# Autodesk Inventor assembly: Drivebase AM14U4 Square 28inx28in v411
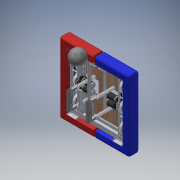
[picture p0: Inventor's stored thumbnail of the model, 180x180]
Saved by Autodesk Inventor 2018 (Build 220112000, 112)
## iProperties
Created: 2020-01-28
Part Number: Drivebase AM14U4 Square 28inx28in v411
Document SubType Name: Assembly
Designer: Weeb No1
Sending System: Autodesk Translation Framework v8.12.0.6
Preprocessor: ST-DEVELOPER v18
Title: /Users/GabG/Documents/GitHub/2020CAD/New Gabriel Shooter/Drivebase AM14U4 Square 28inx28in v41.step
## Documents named in this file (17)
- C:\Users\Weeb No1\Documents\GitHub\2020CAD\Gabriel Fixed Inventor Versions\Drivebase\Main Assembly\Drivebase AM14U4 Square 28inx28in v411.iam
- C:\Users\Weeb No1\Documents\GitHub\2020CAD\Gabriel Fixed Inventor Versions\Drivebase\Part Files\AM14U4 Square Half.iam
- C:\Users\Weeb No1\Documents\GitHub\2020CAD\Gabriel Fixed Inventor Versions\Drivebase\Part Files\AM14U4 Square Half_1.iam
- C:\Users\Weeb No1\Documents\GitHub\2020CAD\Gabriel Fixed Inventor Versions\Drivebase\Part Files\Placeholder Belly Pan.ipt
- C:\Users\Weeb No1\Documents\GitHub\2020CAD\Gabriel Fixed Inventor Versions\Drivebase\Part Files\10-24 Washer.ipt
- C:\Users\Weeb No1\Documents\GitHub\2020CAD\Gabriel Fixed Inventor Versions\Drivebase\Part Files\Bumper Assembly.iam
- C:\Users\Weeb No1\Documents\GitHub\2020CAD\Gabriel Fixed Inventor Versions\Drivebase\Part Files\Bumper Assembly_1.iam
- C:\Users\Weeb No1\Documents\GitHub\2020CAD\Gabriel Fixed Inventor Versions\Drivebase\Part Files\95335A503_METRIC QUICK-RELEASE PIN.ipt
- C:\Users\Weeb No1\Documents\GitHub\2020CAD\Gabriel Fixed Inventor Versions\Drivebase\Part Files\8020 1010 x 19 v2.ipt
- C:\Users\Weeb No1\Documents\GitHub\2020CAD\Gabriel Fixed Inventor Versions\Drivebase\Part Files\8020 1010 x 11 5 v2.ipt
- C:\Users\Weeb No1\Documents\GitHub\2020CAD\Gabriel Fixed Inventor Versions\Drivebase\Part Files\1x2 9in 1_16_ Beam v7.ipt
- C:\Users\Weeb No1\Documents\GitHub\2020CAD\Gabriel Fixed Inventor Versions\Drivebase\Part Files\L-Guesset v1.ipt
- C:\Users\Weeb No1\Documents\GitHub\2020CAD\Gabriel Fixed Inventor Versions\Drivebase\Part Files\L-Bracket v1.ipt
- C:\Users\Weeb No1\Documents\GitHub\2020CAD\Gabriel Fixed Inventor Versions\Drivebase\Part Files\Component52.ipt
- C:\Users\Weeb No1\Documents\GitHub\2020CAD\Gabriel Fixed Inventor Versions\Drivebase\Part Files\8020 1010 x 8 7_8 v6.ipt
- C:\Users\Weeb No1\Documents\GitHub\2020CAD\Gabriel Fixed Inventor Versions\Drivebase\Part Files\am-2986 FR8ZZ Hex Bearing v1.ipt
- C:\Users\Weeb No1\Documents\GitHub\2020CAD\Gabriel Fixed Inventor Versions\Drivebase\Part Files\Clamping_Shaft_Collar_-_1_2_Hex_ID_217-2737 v1.ipt
## Components (59 placed, 16 different names)
1. AM14U4 Square Half:1 [sub-assembly] — Mate:1, Flush:2, Flush:1, Mate:2, Flush:4, Flush:3
2. AM14U4 Square Half_1:1 [sub-assembly]
3. Placeholder Belly Pan:1 — Mate:21, Mate:59, Mate:22, Mate:58
4. 10-24 Washer:1
5. 10-24 Washer:2
6. 10-24 Washer:3
7. 10-24 Washer:4
8. 10-24 Washer:5
9. 10-24 Washer:6
10. 10-24 Washer:7
11. 10-24 Washer:8
12. Bumper Assembly:1 [sub-assembly]
13. Bumper Assembly_1:1 [sub-assembly]
14. 95335A503_METRIC QUICK-RELEASE PIN:1
15. 95335A503_METRIC QUICK-RELEASE PIN:2
16. 95335A503_METRIC QUICK-RELEASE PIN:3
17. 95335A503_METRIC QUICK-RELEASE PIN:4
18. 95335A503_METRIC QUICK-RELEASE PIN:5
19. 95335A503_METRIC QUICK-RELEASE PIN:6
20. 95335A503_METRIC QUICK-RELEASE PIN:7
21. 95335A503_METRIC QUICK-RELEASE PIN:8
22. 95335A503_METRIC QUICK-RELEASE PIN:9
23. 95335A503_METRIC QUICK-RELEASE PIN:10
24. 95335A503_METRIC QUICK-RELEASE PIN:11
25. 95335A503_METRIC QUICK-RELEASE PIN:12
26. 8020 1010 x 19 v2:1 — Mate:1, Flush:2, Flush:1, Flush:17, Mate:20, Mate:19
27. 8020 1010 x 19 v2:2 — Mate:2, Flush:4, Flush:3, Mate:60, Flush:41, Mate:61
28. 8020 1010 x 11 5 v2:1 — Mate:21, Flush:17, Mate:20, Mate:18, Flush:16, Flush:15, Flush:18, Mate:25
29. 8020 1010 x 11 5 v2:2 — Mate:60, Flush:41, Mate:59, Flush:39, Flush:38, Mate:56, Mate:55, Flush:23, Mate:32
30. 8020 1010 x 11 5 v2:3 — Mate:22, Mate:19, Flush:14, Flush:13, Mate:17, Flush:21, Mate:29
31. 1x2 9in 1_16_ Beam v7:1 — Mate:18, Flush:16, Flush:15, Flush:14, Flush:13, Mate:17, Mate:8, Mate:7, Mate:6, Flush:8, Flush:7, Mate:14, Mate:13, Mate:12, Flush:12, Flush:11, Flush:32, Flush:31, Mate:5, Mate:4, Mate:3, Flush:6, Flush:5, Mate:11, Mate:10, Mate:9, Flush:10, Flush:9, Mate:16, Mate:15
32. 8020 1010 x 11 5 v2:4 — Mate:61, Mate:58, Flush:40, Flush:37, Mate:57, Flush:28, Mate:37
33. 1x2 9in 1_16_ Beam v7:2 — Flush:40, Flush:39, Flush:38, Flush:37, Mate:57, Mate:56, Mate:55, Flush:34, Flush:33, Mate:51, Mate:50, Mate:49, Flush:36, Flush:35, Mate:54, Mate:53, Mate:52, Mate:48, Mate:47, Mate:46, Flush:30, Flush:29, Mate:45, Mate:44, Mate:43, Mate:40, Mate:39
34. L-Guesset v1:1 — Flush:18, Mate:25, Flush:19, Mate:27, Mate:26, Mate:24, Mate:23
35. L-Bracket v1:1 — Flush:19, Mate:27, Mate:26, Flush:20, Mate:28
36. L-Guesset v1:2 — Flush:23, Mate:32, Flush:26, Mate:34, Flush:24, Mate:33
37. L-Bracket v1:2 — Flush:26, Mate:34, Flush:25, Mate:35
38. L-Guesset v1:3 — Mate:8, Mate:7, Mate:6, Flush:8, Flush:7
39. L-Guesset v1:4 — Mate:14, Mate:13, Mate:12, Flush:12, Flush:11
40. L-Guesset v1:5 — Flush:34, Flush:33, Mate:51, Mate:50, Mate:49
41. L-Guesset v1:6 — Flush:36, Flush:35, Mate:54, Mate:53, Mate:52
42. L-Guesset v1:7 — Flush:32, Flush:31, Mate:5, Mate:4, Mate:3, Flush:6, Flush:5
43. L-Guesset v1:8 — Mate:11, Mate:10, Mate:9, Flush:10, Flush:9
44. L-Guesset v1:9 — Mate:48, Mate:47, Mate:46
45. L-Guesset v1:10 — Flush:30, Flush:29, Mate:45, Mate:44, Mate:43
46. L-Bracket v1:3
47. L-Bracket v1:4
48. Component52:1
49. L-Guesset v1:11 — Flush:21, Mate:29, Flush:22, Mate:31, Mate:30
50. L-Guesset v1:12 — Flush:28, Mate:37, Flush:27, Mate:38, Mate:36
51. L-Bracket v1:5
52. L-Bracket v1:6
53. L-Bracket v1:7
54. L-Bracket v1:8
55. 8020 1010 x 8 7_8 v6:1 — Flush:27, Mate:38, Mate:36, Flush:25, Mate:35, Flush:24, Mate:33
56. 8020 1010 x 8 7_8 v6:2 — Flush:22, Mate:31, Mate:30, Flush:20, Mate:28, Mate:24, Mate:23
57. am-2986 FR8ZZ Hex Bearing v1:1 — Mate:40, Mate:39, Mate:42, Mate:41
58. Clamping_Shaft_Collar_-_1_2_Hex_ID_217-2737 v1:1 — Mate:42, Mate:41
59. am-2986 FR8ZZ Hex Bearing v1:2 — Mate:16, Mate:15
## Relationships (102: Mate 61, Flush 41)
- Mate:1: AM14U4 Square Half:1 ↔ 8020 1010 x 19 v2:1
- Flush:2 (247.65 mm): AM14U4 Square Half:1 ↔ 8020 1010 x 19 v2:1
- Flush:1: AM14U4 Square Half:1 ↔ 8020 1010 x 19 v2:1
- Mate:2: AM14U4 Square Half:1 ↔ 8020 1010 x 19 v2:2
- Flush:4 (247.65 mm): AM14U4 Square Half:1 ↔ 8020 1010 x 19 v2:2
- Flush:3: AM14U4 Square Half:1 ↔ 8020 1010 x 19 v2:2
- Mate:21: Placeholder Belly Pan:1 ↔ 8020 1010 x 11 5 v2:1
- Flush:17 (9.525 mm): 8020 1010 x 19 v2:1 ↔ 8020 1010 x 11 5 v2:1
- Mate:20: 8020 1010 x 19 v2:1 ↔ 8020 1010 x 11 5 v2:1
- Mate:60: 8020 1010 x 19 v2:2 ↔ 8020 1010 x 11 5 v2:2
- Flush:41 (9.525 mm): 8020 1010 x 19 v2:2 ↔ 8020 1010 x 11 5 v2:2
- Mate:59: Placeholder Belly Pan:1 ↔ 8020 1010 x 11 5 v2:2
- Mate:22: Placeholder Belly Pan:1 ↔ 8020 1010 x 11 5 v2:3
- Mate:19: 8020 1010 x 19 v2:1 ↔ 8020 1010 x 11 5 v2:3
- Mate:18: 8020 1010 x 11 5 v2:1 ↔ 1x2 9in 1_16_ Beam v7:1
- Flush:16: 8020 1010 x 11 5 v2:1 ↔ 1x2 9in 1_16_ Beam v7:1
- Flush:15: 8020 1010 x 11 5 v2:1 ↔ 1x2 9in 1_16_ Beam v7:1
- Flush:14: 8020 1010 x 11 5 v2:3 ↔ 1x2 9in 1_16_ Beam v7:1
- Flush:13: 8020 1010 x 11 5 v2:3 ↔ 1x2 9in 1_16_ Beam v7:1
- Mate:17: 8020 1010 x 11 5 v2:3 ↔ 1x2 9in 1_16_ Beam v7:1
- Mate:61: 8020 1010 x 19 v2:2 ↔ 8020 1010 x 11 5 v2:4
- Mate:58: Placeholder Belly Pan:1 ↔ 8020 1010 x 11 5 v2:4
- Flush:40: 8020 1010 x 11 5 v2:4 ↔ 1x2 9in 1_16_ Beam v7:2
- Flush:39: 8020 1010 x 11 5 v2:2 ↔ 1x2 9in 1_16_ Beam v7:2
- Flush:38: 8020 1010 x 11 5 v2:2 ↔ 1x2 9in 1_16_ Beam v7:2
- Flush:37: 8020 1010 x 11 5 v2:4 ↔ 1x2 9in 1_16_ Beam v7:2
- Mate:57: 8020 1010 x 11 5 v2:4 ↔ 1x2 9in 1_16_ Beam v7:2
- Mate:56: 8020 1010 x 11 5 v2:2 ↔ 1x2 9in 1_16_ Beam v7:2
- Mate:55: 8020 1010 x 11 5 v2:2 ↔ 1x2 9in 1_16_ Beam v7:2
- Flush:18: 8020 1010 x 11 5 v2:1 ↔ L-Guesset v1:1
- Mate:25: 8020 1010 x 11 5 v2:1 ↔ L-Guesset v1:1
- Flush:19: L-Guesset v1:1 ↔ L-Bracket v1:1
- Mate:27: L-Guesset v1:1 ↔ L-Bracket v1:1
- Mate:26: L-Guesset v1:1 ↔ L-Bracket v1:1
- Flush:23: 8020 1010 x 11 5 v2:2 ↔ L-Guesset v1:2
- Mate:32: 8020 1010 x 11 5 v2:2 ↔ L-Guesset v1:2
- Flush:26: L-Guesset v1:2 ↔ L-Bracket v1:2
- Mate:34: L-Guesset v1:2 ↔ L-Bracket v1:2
- Mate:8: 1x2 9in 1_16_ Beam v7:1 ↔ L-Guesset v1:3
- Mate:7: 1x2 9in 1_16_ Beam v7:1 ↔ L-Guesset v1:3
- Mate:6: 1x2 9in 1_16_ Beam v7:1 ↔ L-Guesset v1:3
- Flush:8: 1x2 9in 1_16_ Beam v7:1 ↔ L-Guesset v1:3
- Flush:7: 1x2 9in 1_16_ Beam v7:1 ↔ L-Guesset v1:3
- Mate:14: 1x2 9in 1_16_ Beam v7:1 ↔ L-Guesset v1:4
- Mate:13: 1x2 9in 1_16_ Beam v7:1 ↔ L-Guesset v1:4
- Mate:12: 1x2 9in 1_16_ Beam v7:1 ↔ L-Guesset v1:4
- Flush:12: 1x2 9in 1_16_ Beam v7:1 ↔ L-Guesset v1:4
- Flush:11: 1x2 9in 1_16_ Beam v7:1 ↔ L-Guesset v1:4
- Flush:34: 1x2 9in 1_16_ Beam v7:2 ↔ L-Guesset v1:5
- Flush:33: 1x2 9in 1_16_ Beam v7:2 ↔ L-Guesset v1:5
- Mate:51: 1x2 9in 1_16_ Beam v7:2 ↔ L-Guesset v1:5
- Mate:50: 1x2 9in 1_16_ Beam v7:2 ↔ L-Guesset v1:5
- Mate:49: 1x2 9in 1_16_ Beam v7:2 ↔ L-Guesset v1:5
- Flush:36: 1x2 9in 1_16_ Beam v7:2 ↔ L-Guesset v1:6
- Flush:35: 1x2 9in 1_16_ Beam v7:2 ↔ L-Guesset v1:6
- Mate:54: 1x2 9in 1_16_ Beam v7:2 ↔ L-Guesset v1:6
- Mate:53: 1x2 9in 1_16_ Beam v7:2 ↔ L-Guesset v1:6
- Mate:52: 1x2 9in 1_16_ Beam v7:2 ↔ L-Guesset v1:6
- Flush:32: 1x2 9in 1_16_ Beam v7:1 ↔ L-Guesset v1:7
- Flush:31: 1x2 9in 1_16_ Beam v7:1 ↔ L-Guesset v1:7
- Mate:5: 1x2 9in 1_16_ Beam v7:1 ↔ L-Guesset v1:7
- Mate:4: 1x2 9in 1_16_ Beam v7:1 ↔ L-Guesset v1:7
- Mate:3: 1x2 9in 1_16_ Beam v7:1 ↔ L-Guesset v1:7
- Flush:6: 1x2 9in 1_16_ Beam v7:1 ↔ L-Guesset v1:7
- Flush:5: 1x2 9in 1_16_ Beam v7:1 ↔ L-Guesset v1:7
- Mate:11: 1x2 9in 1_16_ Beam v7:1 ↔ L-Guesset v1:8
- Mate:10: 1x2 9in 1_16_ Beam v7:1 ↔ L-Guesset v1:8
- Mate:9: 1x2 9in 1_16_ Beam v7:1 ↔ L-Guesset v1:8
- Flush:10: 1x2 9in 1_16_ Beam v7:1 ↔ L-Guesset v1:8
- Flush:9: 1x2 9in 1_16_ Beam v7:1 ↔ L-Guesset v1:8
- Mate:48: 1x2 9in 1_16_ Beam v7:2 ↔ L-Guesset v1:9
- Mate:47: 1x2 9in 1_16_ Beam v7:2 ↔ L-Guesset v1:9
- Mate:46: 1x2 9in 1_16_ Beam v7:2 ↔ L-Guesset v1:9
- Flush:30: 1x2 9in 1_16_ Beam v7:2 ↔ L-Guesset v1:10
- Flush:29: 1x2 9in 1_16_ Beam v7:2 ↔ L-Guesset v1:10
- Mate:45: 1x2 9in 1_16_ Beam v7:2 ↔ L-Guesset v1:10
- Mate:44: 1x2 9in 1_16_ Beam v7:2 ↔ L-Guesset v1:10
- Mate:43: 1x2 9in 1_16_ Beam v7:2 ↔ L-Guesset v1:10
- Flush:21: 8020 1010 x 11 5 v2:3 ↔ L-Guesset v1:11
- Mate:29: 8020 1010 x 11 5 v2:3 ↔ L-Guesset v1:11
- Flush:28: 8020 1010 x 11 5 v2:4 ↔ L-Guesset v1:12
- Mate:37: 8020 1010 x 11 5 v2:4 ↔ L-Guesset v1:12
- Flush:27: L-Guesset v1:12 ↔ 8020 1010 x 8 7_8 v6:1
- Mate:38: L-Guesset v1:12 ↔ 8020 1010 x 8 7_8 v6:1
- Mate:36: L-Guesset v1:12 ↔ 8020 1010 x 8 7_8 v6:1
- Flush:25: L-Bracket v1:2 ↔ 8020 1010 x 8 7_8 v6:1
- Mate:35: L-Bracket v1:2 ↔ 8020 1010 x 8 7_8 v6:1
- Flush:24: L-Guesset v1:2 ↔ 8020 1010 x 8 7_8 v6:1
- Mate:33: L-Guesset v1:2 ↔ 8020 1010 x 8 7_8 v6:1
- Flush:22: L-Guesset v1:11 ↔ 8020 1010 x 8 7_8 v6:2
- Mate:31: L-Guesset v1:11 ↔ 8020 1010 x 8 7_8 v6:2
- Mate:30: L-Guesset v1:11 ↔ 8020 1010 x 8 7_8 v6:2
- Flush:20: L-Bracket v1:1 ↔ 8020 1010 x 8 7_8 v6:2
- Mate:28: L-Bracket v1:1 ↔ 8020 1010 x 8 7_8 v6:2
- Mate:24: L-Guesset v1:1 ↔ 8020 1010 x 8 7_8 v6:2
- Mate:23: L-Guesset v1:1 ↔ 8020 1010 x 8 7_8 v6:2
- Mate:40: 1x2 9in 1_16_ Beam v7:2 ↔ am-2986 FR8ZZ Hex Bearing v1:1
- Mate:39: 1x2 9in 1_16_ Beam v7:2 ↔ am-2986 FR8ZZ Hex Bearing v1:1
- Mate:42: am-2986 FR8ZZ Hex Bearing v1:1 ↔ Clamping_Shaft_Collar_-_1_2_Hex_ID_217-2737 v1:1
- Mate:41: am-2986 FR8ZZ Hex Bearing v1:1 ↔ Clamping_Shaft_Collar_-_1_2_Hex_ID_217-2737 v1:1
- Mate:16: 1x2 9in 1_16_ Beam v7:1 ↔ am-2986 FR8ZZ Hex Bearing v1:2
- Mate:15: 1x2 9in 1_16_ Beam v7:1 ↔ am-2986 FR8ZZ Hex Bearing v1:2
